# Autodesk Inventor assembly: assembledLinkage
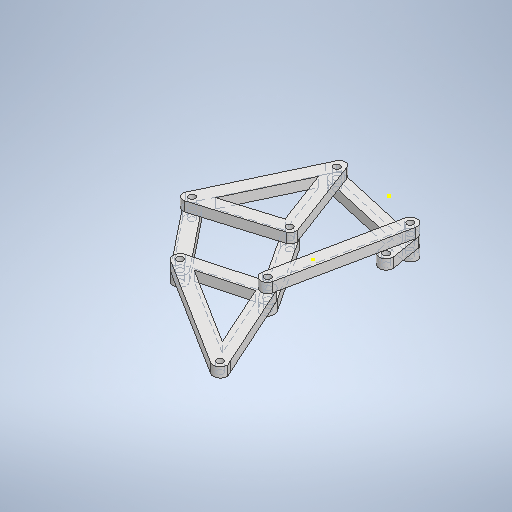
[picture p0: Inventor's stored thumbnail of the model, 512x512]
Saved by Autodesk Inventor 2025.1 (Build 291241020, 241B)
## iProperties
Created: 2025-05-24
Part Number: assembledLinkage
Document SubType Name: Assembly
Designer: omiye
Author: omiye
## Documents named in this file (9)
- C:\Projects\Arduino\strandbeest\assembledLinkage.iam
- C:\Projects\Arduino\strandbeest\f.ipt
- C:\Projects\Arduino\strandbeest\k.ipt
- C:\Projects\Arduino\strandbeest\c.ipt
- C:\Projects\Arduino\strandbeest\bde.ipt
- C:\Projects\Arduino\strandbeest\ghi.ipt
- C:\Projects\Arduino\strandbeest\m.ipt
- C:\Projects\Arduino\strandbeest\j.ipt
- C:\Projects\Arduino\strandbeest\connector.ipt
## Components (8 placed, 8 different names)
1. f:1 — Mate:13, Mate:14, Mate:25, Mate:26
2. k:1 — Mate:2, Mate:5, Mate:16, Mate:23, Mate:27
3. c:1 — Mate:15, Mate:16, Mate:24, Mate:28, Mate:29
4. bde:1 — Mate:7, Mate:13, Mate:15, Flush:1, Mate:25, Mate:26
5. ghi:1 — Mate:5, Mate:14, Mate:23, Mate:24, Flush:1
6. m:1 — Mate:2, Mate:3, Mate:21, Mate:22, Mate:27
7. j:1 — Mate:3, Mate:7, Mate:22
8. connector:1 — Mate:21, Mate:28, Mate:29
## Relationships (18: Mate 17, Flush 1)
- Mate:2: k:1 ↔ m:1
- Mate:3: m:1 ↔ j:1
- Mate:5: k:1 ↔ ghi:1
- Mate:7: bde:1 ↔ j:1
- Mate:13: f:1 ↔ bde:1
- Mate:14: f:1 ↔ ghi:1
- Mate:15: c:1 ↔ bde:1
- Mate:16: k:1 ↔ c:1
- Mate:21: m:1 ↔ connector:1
- Mate:22: m:1 ↔ j:1
- Mate:23: k:1 ↔ ghi:1
- Mate:24: c:1 ↔ ghi:1
- Flush:1: bde:1 ↔ ghi:1
- Mate:25: f:1 ↔ bde:1
- Mate:26: f:1 ↔ bde:1
- Mate:27: k:1 ↔ m:1
- Mate:28: c:1 ↔ connector:1
- Mate:29: c:1 ↔ connector:1
